# Autodesk Inventor assembly: WallEAssembly
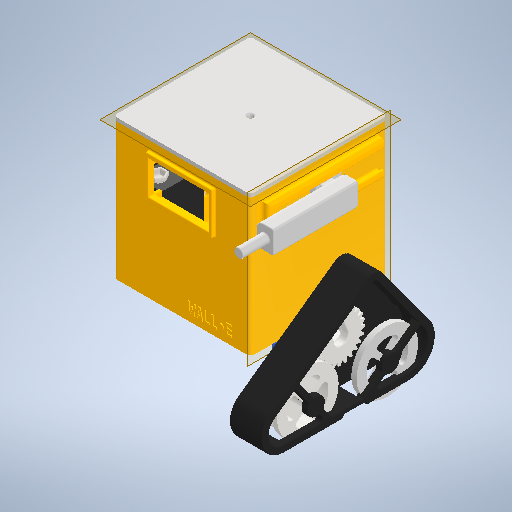
[picture p0: Inventor's stored thumbnail of the model, 512x512]
Saved by Autodesk Inventor 2025.2 (Build 292293000, 293)
## iProperties
Created: 2025-01-25
Part Number: WallEAssembly
Document SubType Name: Assembly
Designer: andre
Author: andre
## Documents named in this file (13)
- C:\Users\andre\Documents\GitHub\Handshake\Hardware\Proto2-WallE\WallEAssembly.iam
- C:\Users\andre\Documents\GitHub\Handshake\Hardware\Proto2-WallE\WallEBody.ipt
- C:\Users\andre\Documents\GitHub\Handshake\Hardware\Common\PCBModel.ipt
- C:\Users\andre\Documents\GitHub\Handshake\Hardware\Common\Battery_9V\Battery_9V\Battery_9V.ipt
- C:\Users\andre\Documents\GitHub\Handshake\Hardware\Proto2-WallE\TreadAssembly.iam
- C:\Users\andre\Documents\GitHub\Handshake\Hardware\Common\Servo Motor SG90.ipt
- C:\Users\andre\Documents\GitHub\Handshake\Hardware\Proto2-WallE\ BodyLid.ipt
- C:\Users\andre\Documents\GitHub\Handshake\Hardware\Proto2-WallE\WheelBetter.ipt
- C:\Users\andre\Documents\GitHub\Handshake\Hardware\Proto2-WallE\WallEAssembly\Design Accelerator\Spur Gear21.ipt
- C:\Users\andre\Documents\GitHub\Handshake\Hardware\Proto2-WallE\WallEAssembly\Design Accelerator\Spur Gear11.ipt
- C:\Users\andre\Documents\GitHub\Handshake\Hardware\Proto2-WallE\Arm.ipt
- C:\Users\andre\Documents\GitHub\Handshake\Hardware\Proto2-WallE\ArmLength.ipt
- C:\Users\andre\Documents\GitHub\Handshake\Hardware\Proto2-WallE\BodyLid.ipt
## Components (11 placed, 11 different names)
1. WallEBody:1 — Mate:1, Angle:1, Mate:2, Mate:3, Mate:4, Angle:2, Mate:5, Mate:6, Mate:8, Mate:9, Flush:1, Flush:2, Flush:3, Flush:4
2. PCBModel:1 — Mate:1, Angle:1, Mate:2
3. Battery_9V:1 — Mate:3, Mate:8
4. TreadAssembly:1 [sub-assembly] — Mate:4, Angle:2, Mate:5, Mate:6, Mate:7, Mate:13, Mate:14, Mate:15, Mate:18
5. Servo Motor SG90:1 — Mate:7, Mate:9, Mate:13, Mate:16, Mate:17
6. BodyLid:1 — Flush:1, Flush:2
7. WheelBetter:1 — Mate:14
8. Spur Gear2:1 — Mate:16, Mate:17
9. Spur Gear1:1 — Mate:15, Mate:18
10. Arm:1 — Flush:3, Flush:4, Mate:19, Angle:3
11. ArmLength:1 — Mate:19, Angle:3
## Relationships (23: Mate 16, Flush 4, Angle 3)
- Mate:1 (2.3 mm): WallEBody:1 ↔ PCBModel:1
- Angle:1 (0 deg): WallEBody:1 ↔ PCBModel:1
- Mate:2: WallEBody:1 ↔ PCBModel:1
- Mate:3: WallEBody:1 ↔ Battery_9V:1
- Mate:4: WallEBody:1 ↔ TreadAssembly:1
- Angle:2 (0 deg): WallEBody:1 ↔ TreadAssembly:1
- Mate:5: WallEBody:1 ↔ TreadAssembly:1
- Mate:6: WallEBody:1 ↔ TreadAssembly:1
- Mate:7: TreadAssembly:1 ↔ Servo Motor SG90:1
- Mate:8: WallEBody:1 ↔ Battery_9V:1
- Mate:9: WallEBody:1 ↔ Servo Motor SG90:1
- Flush:1: WallEBody:1 ↔ BodyLid:1
- Flush:2: WallEBody:1 ↔ BodyLid:1
- Mate:13: TreadAssembly:1 ↔ Servo Motor SG90:1
- Mate:14: TreadAssembly:1 ↔ WheelBetter:1
- Mate:15: TreadAssembly:1 ↔ Spur Gear1:1
- Mate:16: Servo Motor SG90:1 ↔ Spur Gear2:1
- Mate:17: Servo Motor SG90:1 ↔ Spur Gear2:1
- Mate:18: TreadAssembly:1 ↔ Spur Gear1:1
- Flush:3: WallEBody:1 ↔ Arm:1
- Flush:4: WallEBody:1 ↔ Arm:1
- Mate:19: Arm:1 ↔ ArmLength:1
- Angle:3 (0 deg): Arm:1 ↔ ArmLength:1
